# Autodesk Inventor assembly: BoronProbe
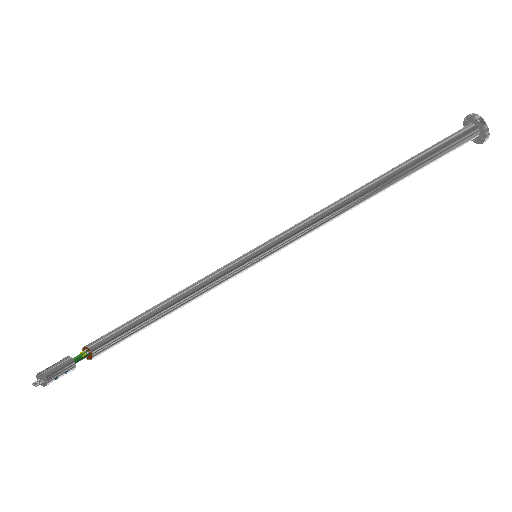
[picture p0: Inventor's stored thumbnail of the model, 512x512]
Saved by Autodesk Inventor 2026.2 (Build 302298000, 298)
## iProperties
Created: 2024-05-30
Part Number: BoronProbe
Document SubType Name: Assembly
Designer: kuzmin
Author: kuzmin
## Documents named in this file (10)
- D:\repos\PIHTI\BoronProbe\BoronProbe.iam
- D:\repos\PIHTI\PALP\CF34-nipples-for-PALP\ICF34_70mmNipple.iam
- D:\repos\PIHTI\PALP\Prototype-PALP-ring-to-pipe-adapter_4mm.ipt
- D:\repos\PIHTI\ContentCenter\Ceramics\Electric-feeds\feed_4.ipt
- D:\repos\PIHTI\PALP\Prototype-PALP-pipe-neck-straight.ipt
- D:\repos\PIHTI\PALP\Prototype-PALP-CF34-flange.ipt
- D:\repos\PIHTI\PALP\wire_connector.ipt
- D:\repos\PIHTI\PALP\Probe-clamp-v1.iam
- D:\repos\PIHTI\BoronProbe\BoronProbePipe.iam
- D:\repos\PIHTI\BoronProbe\BoronProbeHead.iam
## Components (12 placed, 9 different names)
1. BoronProbePipe:1 [sub-assembly]
2. ICF34_70mmNipple:1 [sub-assembly] — 回転:2, メイト:4, メイト:15, リジッド:9
3. Prototype-PALP-ring-to-pipe-adapter_4mm:1 — 回転:6, フラッシュ:1, リジッド:7, リジッド:8
4. feed_4:1 — 円柱状:1, リジッド:8
5. feed_4:2 — 円柱状:2, リジッド:7
6. Prototype-PALP-pipe-neck-straight:1 — 回転:6, リジッド:4
7. Prototype-PALP-CF34-flange:1 — リジッド:4, 回転:2, メイト:4, メイト:5
8. wire_connector:1 — 円柱状:1
9. wire_connector:2 — 円柱状:2
10. Probe-clamp-v1:1 [sub-assembly] — メイト:16
11. Probe-clamp-v1:2 [sub-assembly] — メイト:15, メイト:16
12. BoronProbeHead:1 [sub-assembly] — リジッド:9
## Relationships (18: Mate 8, WeldJoint 4, RevoluteJoint 3, CylindricalJoint 2, Flush 1)
- [Mate]: BoronProbePipe:1 ↔ ICF34_70mmNipple:1
- [Mate]: BoronProbePipe:1 ↔ Prototype-PALP-ring-to-pipe-adapter_4mm:1
- [RevoluteJoint]: BoronProbePipe:1 ↔ Prototype-PALP-ring-to-pipe-adapter_4mm:1
- 回転:6 [RevoluteJoint]: Prototype-PALP-ring-to-pipe-adapter_4mm:1 ↔ Prototype-PALP-pipe-neck-straight:1
- リジッド:4 [WeldJoint]: Prototype-PALP-pipe-neck-straight:1 ↔ Prototype-PALP-CF34-flange:1
- 回転:2 [RevoluteJoint]: ICF34_70mmNipple:1 ↔ Prototype-PALP-CF34-flange:1
- メイト:4 [Mate]: ICF34_70mmNipple:1 ↔ Prototype-PALP-CF34-flange:1
- フラッシュ:1 [Flush]: Prototype-PALP-ring-to-pipe-adapter_4mm:1
- メイト:5 [Mate]: Prototype-PALP-CF34-flange:1
- [Mate]: ICF34_70mmNipple:1 ↔ Probe-clamp-v1:1
- [Mate]: Probe-clamp-v1:1
- 円柱状:1 [CylindricalJoint]: feed_4:1 ↔ wire_connector:1
- 円柱状:2 [CylindricalJoint]: feed_4:2 ↔ wire_connector:2
- リジッド:7 [WeldJoint]: Prototype-PALP-ring-to-pipe-adapter_4mm:1 ↔ feed_4:2
- リジッド:8 [WeldJoint]: Prototype-PALP-ring-to-pipe-adapter_4mm:1 ↔ feed_4:1
- メイト:15 [Mate]: ICF34_70mmNipple:1 ↔ Probe-clamp-v1:2
- メイト:16 [Mate]: Probe-clamp-v1:1 ↔ Probe-clamp-v1:2
- リジッド:9 [WeldJoint]: ICF34_70mmNipple:1 ↔ BoronProbeHead:1
